# Autodesk Inventor assembly: shooter
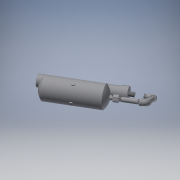
[picture p0: Inventor's stored thumbnail of the model, 180x180]
Saved by Autodesk Inventor 2018 (Build 220112000, 112)
## iProperties
Created: 2017-05-02
Part Number: shooter
Document SubType Name: Assembly
Designer: gsegs
Author: gsegs
## Documents named in this file (7)
- C:\Users\gsegs\OneDrive\Documents\GitHub\RoboEaglesCad2018\shooter.iam
- C:\Users\gsegs\OneDrive\Documents\GitHub\RoboEaglesCad2018\6in pipe.ipt
- C:\Users\gsegs\OneDrive\Documents\GitHub\RoboEaglesCad2018\90 angle pipe.ipt
- C:\Users\gsegs\OneDrive\Documents\GitHub\RoboEaglesCad2018\90 angle pipe 2.ipt
- C:\Users\gsegs\OneDrive\Documents\GitHub\RoboEaglesCad2018\adapter.ipt
- C:\Users\gsegs\OneDrive\Documents\GitHub\RoboEaglesCad2018\long pipe.ipt
- C:\Users\gsegs\OneDrive\Documents\GitHub\RoboEaglesCad2018\air canister.ipt
## Components (7 placed, 6 different names)
1. 6in pipe:1 — Mate:5, Mate:6, Mate:9
2. 6in pipe:2 — Mate:1, Mate:2, Mate:10
3. 90 angle pipe:1 — Mate:2, Mate:3, Mate:4, Mate:5, Mate:10
4. 90 angle pipe 2:1 — Mate:1, Mate:3, Mate:7, Mate:8
5. adapter:1 — Mate:4, Mate:6, Mate:9, Mate:11, Mate:12
6. long pipe:1 — Mate:7, Mate:8, Angle:1
7. air canister:1 — Mate:11, Angle:1, Mate:12
## Relationships (13: Mate 12, Angle 1)
- Mate:1: 6in pipe:2 ↔ 90 angle pipe 2:1
- Mate:2: 6in pipe:2 ↔ 90 angle pipe:1
- Mate:3 (133.35 mm): 90 angle pipe:1 ↔ 90 angle pipe 2:1
- Mate:4 (134.9375 mm): 90 angle pipe:1 ↔ adapter:1
- Mate:5: 6in pipe:1 ↔ 90 angle pipe:1
- Mate:6: 6in pipe:1 ↔ adapter:1
- Mate:7 (114.3 mm): 90 angle pipe 2:1 ↔ long pipe:1
- Mate:8: 90 angle pipe 2:1 ↔ long pipe:1
- Mate:9 (25.4 mm): 6in pipe:1 ↔ adapter:1
- Mate:10 (12.7 mm): 6in pipe:2 ↔ 90 angle pipe:1
- Mate:11 (8.89 mm): adapter:1 ↔ air canister:1
- Angle:1 (0 deg): long pipe:1 ↔ air canister:1
- Mate:12: adapter:1 ↔ air canister:1
